# Autodesk Inventor assembly: full_assembly
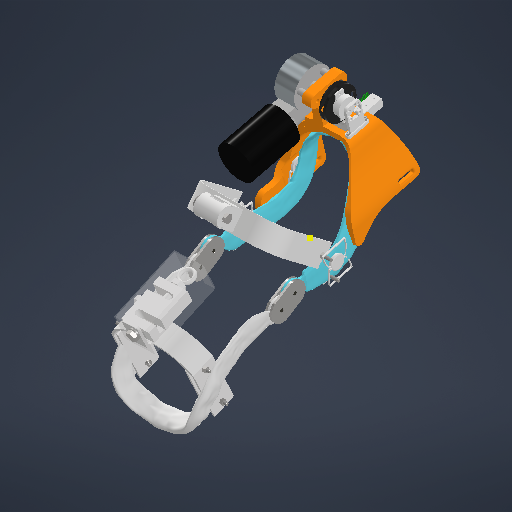
[picture p0: Inventor's stored thumbnail of the model, 512x512]
Saved by Autodesk Inventor 2025.2 (Build 292293000, 293)
## iProperties
Created: 2025-02-17
Part Number: full_assembly
Document SubType Name: Assembly
Designer: email
Author: email
## Documents named in this file (5)
- C:\Shared\alex-bartella-schoolwork\4tb6\4TB6-repo\CAD_Model\thigh_mount_2\full_assembly.iam
- C:\Shared\alex-bartella-schoolwork\4tb6\4TB6-repo\CAD_Model\thigh_mount_2\mount3.iam
- C:\Shared\alex-bartella-schoolwork\4tb6\4TB6-repo\CAD_Model\thigh_mount_2\hinge.ipt
- C:\Shared\alex-bartella-schoolwork\4tb6\4TB6-repo\CAD_Model\thigh_mount_2\rivet.ipt
- C:\Shared\alex-bartella-schoolwork\4tb6\4TB6-repo\CAD_Model\thigh_mount_2\shin_assembly.iam
## Components (10 placed, 4 different names)
1. mount3:1 [sub-assembly] — Mate:1, Mate:5, Mate:9, Mate:10, Mate:12, Mate:18, Flush:5
2. hinge:1 — Mate:3, Mate:4, Mate:5, Flush:1, Flush:2, Mate:20
3. hinge:2 — Mate:7, Mate:8, Mate:9
4. hinge:3 — Mate:16, Mate:17, Mate:18
5. hinge:4 — Mate:12, Mate:14, Mate:15, Flush:3, Flush:4
6. rivet:1 — Mate:1, Mate:3, Flush:1, Mate:7
7. rivet:2 — Mate:4, Flush:2, Mate:8, Mate:19
8. rivet:3 — Mate:10, Mate:14, Flush:3, Mate:16
9. rivet:4 — Mate:15, Flush:4, Mate:17, Mate:21
10. shin_assembly:1 [sub-assembly] — Mate:19, Mate:20, Mate:21, Flush:5
## Relationships (22: Mate 17, Flush 5)
- Mate:1: mount3:1 ↔ rivet:1
- Mate:3: hinge:1 ↔ rivet:1
- Mate:4: hinge:1 ↔ rivet:2
- Mate:5: mount3:1 ↔ hinge:1
- Flush:1: hinge:1 ↔ rivet:1
- Flush:2: hinge:1 ↔ rivet:2
- Mate:7: hinge:2 ↔ rivet:1
- Mate:8: hinge:2 ↔ rivet:2
- Mate:9: mount3:1 ↔ hinge:2
- Mate:10: mount3:1 ↔ rivet:3
- Mate:12: mount3:1 ↔ hinge:4
- Mate:14: hinge:4 ↔ rivet:3
- Mate:15: hinge:4 ↔ rivet:4
- Flush:3: hinge:4 ↔ rivet:3
- Flush:4: hinge:4 ↔ rivet:4
- Mate:16: hinge:3 ↔ rivet:3
- Mate:17: hinge:3 ↔ rivet:4
- Mate:18: mount3:1 ↔ hinge:3
- Mate:19: rivet:2 ↔ shin_assembly:1
- Mate:20: hinge:1 ↔ shin_assembly:1
- Mate:21: rivet:4 ↔ shin_assembly:1
- Flush:5: mount3:1 ↔ shin_assembly:1
